# Autodesk Inventor assembly: аккумулятор 21700
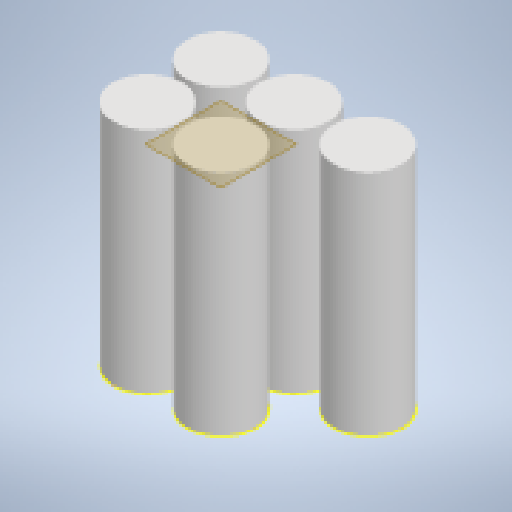
[picture p0: Inventor's stored thumbnail of the model, 512x512]
Saved by Autodesk Inventor 2024.2 (Build 282272000, 272)
## iProperties
Created: 2025-10-05
Part Number: аккумулятор 21700
Document SubType Name: Assembly
Designer: katya_notebook
Author: katya_notebook
## Documents named in this file (2)
- C:\dog\fox\аккумулятор 21700.iam
- C:\dog\fox\21700.ipt
## Components (5 placed, 1 different names)
1. 21700:2 — Совмещение:3, Совмещение:4, Совмещение:6, Совмещение:7, Заподлицо:1
2. 21700:3 — Совмещение:3, Совмещение:5, Совмещение:7
3. 21700:4 — Совмещение:2, Совмещение:8
4. 21700:5 — Совмещение:1, Совмещение:4, Совмещение:6, Совмещение:8
5. 21700:6 — Совмещение:1, Совмещение:2, Совмещение:5
## Relationships (9: Mate 8, Flush 1)
- Совмещение:1 [Mate]: 21700:5 ↔ 21700:6
- Совмещение:2 [Mate]: 21700:4 ↔ 21700:6
- Совмещение:3 [Mate]: 21700:2 ↔ 21700:3
- Совмещение:4 [Mate]: 21700:2 ↔ 21700:5
- Совмещение:5 [Mate]: 21700:3 ↔ 21700:6
- Совмещение:6 [Mate] (22.5 mm): 21700:2 ↔ 21700:5
- Совмещение:7 [Mate] (22.5 mm): 21700:2 ↔ 21700:3
- Совмещение:8 [Mate] (22.5 mm): 21700:4 ↔ 21700:5
- Заподлицо:1 [Flush]: 21700:2
